# Autodesk Inventor assembly: MotorMountAssembly
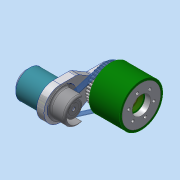
[picture p0: Inventor's stored thumbnail of the model, 180x180]
Saved by Autodesk Inventor 2015 SP1 (Build 190203100, 203)
## iProperties
Created: 2015-06-16
Part Number: MotorMountAssembly
Document SubType Name: Assembly
Designer: YOUR_NAME_HERE
Author: YOUR_NAME_HERE
## Documents named in this file (10)
- C:\Users\Rahul\Electric Skateboard\Electric Skateboard CAD\MotorMountAssembly.iam
- C:\Users\Rahul\Electric Skateboard\Electric Skateboard CAD\MotorMountingPlate.ipt
- C:\Users\Rahul\Electric Skateboard\Electric Skateboard CAD\16T_5mm_a_6a25m016df0906.ipt
- C:\Users\Rahul\Electric Skateboard\Electric Skateboard CAD\TurnigySK3_Mock.ipt
- C:\Users\Rahul\Electric Skateboard\Electric Skateboard CAD\40T_5mm_a_6l25m040sf0908_modified.ipt
- C:\Users\Rahul\Electric Skateboard\Electric Skateboard CAD\TimingBelt.ipt
- C:\Users\Rahul\Electric Skateboard\Electric Skateboard CAD\Imported Components\suspension_assy\wheel_assy_modifiedwheel.iam
- C:\Users\Rahul\Electric Skateboard\Electric Skateboard CAD\TruckBushing.ipt
- C:\Users\Rahul\Electric Skateboard\Electric Skateboard CAD\WheelPlate.ipt
- C:\Users\Rahul\Electric Skateboard\Electric Skateboard CAD\PulleyCover.ipt
## Components (9 placed, 9 different names)
1. MotorMountingPlate:1 — Mate:2, Mate:5, Mate:6, Mate:12, Mate:15, Mate:16, Angle:1, Flush:3
2. 16T_5mm_a_6a25m016df0906:1 — Mate:2, Flush:1, Mate:7, Mate:11
3. TurnigySK3_Mock:1 — Mate:5, Mate:11, Mate:15
4. 40T_5mm_a_6l25m040sf0908_modified:1 — Flush:1, Mate:6, Mate:8, Mate:9, Mate:13, Mate:14, Flush:2
5. TimingBelt:1 — Mate:7, Mate:8, Mate:9
6. wheel_assy_modifiedwheel:1 [sub-assembly] — Mate:12, Mate:13, Mate:14, Mate:17, Mate:18, Mate:19
7. TruckBushing:1 — Mate:16, Flush:2
8. WheelPlate:1 — Mate:17, Mate:18, Mate:19
9. PulleyCover:1 — Angle:1, Flush:3
## Relationships (19: Mate 15, Flush 3, Angle 1)
- Mate:2: MotorMountingPlate:1 ↔ 16T_5mm_a_6a25m016df0906:1
- Mate:5: MotorMountingPlate:1 ↔ TurnigySK3_Mock:1
- Flush:1: 16T_5mm_a_6a25m016df0906:1 ↔ 40T_5mm_a_6l25m040sf0908_modified:1
- Mate:6: MotorMountingPlate:1 ↔ 40T_5mm_a_6l25m040sf0908_modified:1
- Mate:7: 16T_5mm_a_6a25m016df0906:1 ↔ TimingBelt:1
- Mate:8: 40T_5mm_a_6l25m040sf0908_modified:1 ↔ TimingBelt:1
- Mate:9: 40T_5mm_a_6l25m040sf0908_modified:1 ↔ TimingBelt:1
- Mate:11: 16T_5mm_a_6a25m016df0906:1 ↔ TurnigySK3_Mock:1
- Mate:12: MotorMountingPlate:1 ↔ wheel_assy_modifiedwheel:1
- Mate:13: 40T_5mm_a_6l25m040sf0908_modified:1 ↔ wheel_assy_modifiedwheel:1
- Mate:14: 40T_5mm_a_6l25m040sf0908_modified:1 ↔ wheel_assy_modifiedwheel:1
- Mate:15: MotorMountingPlate:1 ↔ TurnigySK3_Mock:1
- Mate:16: MotorMountingPlate:1 ↔ TruckBushing:1
- Flush:2: 40T_5mm_a_6l25m040sf0908_modified:1 ↔ TruckBushing:1
- Mate:17: wheel_assy_modifiedwheel:1 ↔ WheelPlate:1
- Mate:18: wheel_assy_modifiedwheel:1 ↔ WheelPlate:1
- Mate:19: wheel_assy_modifiedwheel:1 ↔ WheelPlate:1
- Angle:1 (180 deg): MotorMountingPlate:1 ↔ PulleyCover:1
- Flush:3: MotorMountingPlate:1 ↔ PulleyCover:1
